# Autodesk Inventor assembly: Blog and Peg
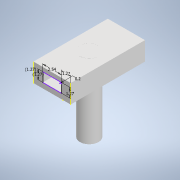
[picture p0: Inventor's stored thumbnail of the model, 180x180]
Saved by Autodesk Inventor 2020.2 (Build 242310000, 310)
## iProperties
Created: 2020-04-17
Part Number: Blog and Peg
Document SubType Name: Assembly
Designer: Tanana
Author: Tanana
## Documents named in this file (3)
- D:\OneDrive - UNSW\CAD Files\Begining 1st project\Blog and Peg.iam
- D:\OneDrive - UNSW\CAD Files\Begining 1st project\Block.ipt
- D:\OneDrive - UNSW\CAD Files\Begining 1st project\Peg.ipt
## Components (2 placed, 2 different names)
1. Block:1 — Mate:1, Flush:1
2. Peg:1 — Mate:1, Flush:1
## Relationships (2: Mate 1, Flush 1)
- Mate:1: Block:1 ↔ Peg:1
- Flush:1: Block:1 ↔ Peg:1
